# Autodesk Inventor assembly: BG301_trajan20_21
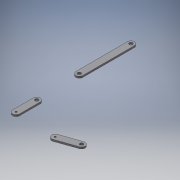
[picture p0: Inventor's stored thumbnail of the model, 180x180]
Saved by Autodesk Inventor 2022.2 (Build 262287000, 287)
## iProperties
Company: HTBLA Kaindorf
RuleStatus: InUse
Created: 2022-08-22
Part Number: BG301_trajan20_21
Project: Zeichenmaschine_v2
Material: Generisch
Description: gelenke
Document SubType Name: Assembly
Designer: trajan20
AfterDocNew0: iProperties-Editor_aufrufen
Author: jan
Keywords: 2021
## Documents named in this file (3)
- C:\Users\jan\Documents\DrawMachine\DrawMachineConstruction\Projekt\Zeichenmaschine_v2\BG301_trajan20_21_Zeichenmaschine_v2_gelenke.iam
- C:\Users\jan\Documents\DrawMachine\DrawMachineConstruction\Projekt\Zeichenmaschine_v2\BT301_trajan20_21_Zeichenmaschine_v2_gelenk 1.ipt
- C:\Users\jan\Documents\DrawMachine\DrawMachineConstruction\Projekt\Zeichenmaschine_v2\BT301_trajan20_21_Zeichenmaschine_v2_gelenk a.ipt
## Components (3 placed, 2 different names)
1. BT301_trajan20_21_Zeichenmaschine_v2_gelenk 1:1 — Passend:1, Fluchtend:1
2. BT301_trajan20_21_Zeichenmaschine_v2_gelenk a:1
3. BT301_trajan20_21_Zeichenmaschine_v2_gelenk 1:2 — Passend:1, Fluchtend:1
## Relationships (2: Mate 1, Flush 1)
- Passend:1 [Mate] (120 mm): BT301_trajan20_21_Zeichenmaschine_v2_gelenk 1:1 ↔ BT301_trajan20_21_Zeichenmaschine_v2_gelenk 1:2
- Fluchtend:1 [Flush]: BT301_trajan20_21_Zeichenmaschine_v2_gelenk 1:1 ↔ BT301_trajan20_21_Zeichenmaschine_v2_gelenk 1:2
